# Autodesk Inventor assembly: ROBOT
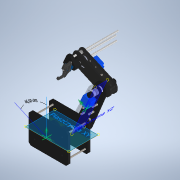
[picture p0: Inventor's stored thumbnail of the model, 180x180]
Saved by Autodesk Inventor 2021 (Build 250183000, 183)
## iProperties
Created: 2021-07-30
Part Number: ROBOT
Description: STEP AP214
Document SubType Name: Assembly
Designer: Janusz
Sending System: SolidWorks 2018
Preprocessor: SwSTEP 2.0
Title: ROBOT.STEP
Revision Number: ANY
## Documents named in this file (7)
- D:\ROBOT\ROBOT.iam
- D:\ROBOT\Podstawa.iam
- D:\ROBOT\Ramie_z.iam
- D:\ROBOT\Przed_Ramie.iam
- D:\ROBOT\Wal_1.iam
- D:\ROBOT\Wal_2.iam
- D:\ROBOT\Chwytak.iam
## Components (6 placed, 6 different names)
1. Podstawa_1 [sub-assembly] — Zestawiające:1, Zestawiające:3, J1, Równoległe:1
2. Ramie_z_2 [sub-assembly] — Zestawiające:1, Zestawiające:2, Zestawiające:4, Zestawiające:5, Zestawiające:6, J2, J1
3. Przed_Ramie_3 [sub-assembly] — Zestawiające:5, Zestawiające:6, Zestawiające:7, Zestawiające:8, Zestawiające:11, Zestawiające:12, J2
4. Wal_1_4 [sub-assembly] — Zestawiające:2, Zestawiające:3, Zestawiające:4
5. Wal_2_5 [sub-assembly] — Zestawiające:7, Zestawiające:8
6. Chwytak_6 [sub-assembly] — Zestawiające:11, Zestawiające:12
## Relationships (13: Mate 10, Angle 2, Flush 1)
- Zestawiające:1 [Mate]: Podstawa_1 ↔ Ramie_z_2
- Zestawiające:2 [Mate]: Ramie_z_2 ↔ Wal_1_4
- Zestawiające:3 [Mate]: Podstawa_1 ↔ Wal_1_4
- Zestawiające:4 [Mate]: Ramie_z_2 ↔ Wal_1_4
- Zestawiające:5 [Mate]: Ramie_z_2 ↔ Przed_Ramie_3
- Zestawiające:6 [Mate]: Ramie_z_2 ↔ Przed_Ramie_3
- Zestawiające:7 [Mate]: Przed_Ramie_3 ↔ Wal_2_5
- Zestawiające:8 [Mate]: Przed_Ramie_3 ↔ Wal_2_5
- Zestawiające:11 [Mate]: Przed_Ramie_3 ↔ Chwytak_6
- Zestawiające:12 [Mate]: Przed_Ramie_3 ↔ Chwytak_6
- J2 [Angle] (90 deg): Ramie_z_2 ↔ Przed_Ramie_3
- J1 [Angle] (66 deg): Podstawa_1 ↔ Ramie_z_2
- Równoległe:1 [Flush] (-75 mm): Podstawa_1
